# Autodesk Inventor assembly: Bridge
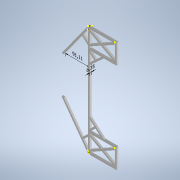
[picture p0: Inventor's stored thumbnail of the model, 180x180]
Saved by Autodesk Inventor 2020.1 (Build 241239000, 239)
## iProperties
Created: 2020-02-04
Part Number: Bridge
Document SubType Name: Assembly
Designer: super
Author: super
## Documents named in this file (8)
- C:\Users\super\Desktop\Giovanni\Science\3D Models\Autodesk-Inventor\Projects\FAS\Bridge.iam
- C:\Users\super\Desktop\Giovanni\Science\3D Models\Autodesk-Inventor\Projects\FAS\BottomBottom.ipt
- C:\Users\super\Desktop\Giovanni\Science\3D Models\Autodesk-Inventor\Projects\FAS\BottomDiagonalSupport.ipt
- C:\Users\super\Desktop\Giovanni\Science\3D Models\Autodesk-Inventor\Projects\FAS\BottomSquareSupport.ipt
- C:\Users\super\Desktop\Giovanni\Science\3D Models\Autodesk-Inventor\Projects\FAS\InnerDiagonalSupport.ipt
- C:\Users\super\Desktop\Giovanni\Science\3D Models\Autodesk-Inventor\Projects\FAS\Main.ipt
- C:\Users\super\Desktop\Giovanni\Science\3D Models\Autodesk-Inventor\Projects\FAS\UpperExteriorDiagonal.ipt
- C:\Users\super\Desktop\Giovanni\Science\3D Models\Autodesk-Inventor\Projects\FAS\UpperMiniSupport.ipt
## Components (19 placed, 7 different names)
1. BottomBottom:1 — Mate:1, Flush:1, Flush:2, Flush:3, Mate:2, Flush:4, Mate:3, Flush:5, Mate:4, Mate:5, Flush:6, Flush:15, Mate:12
2. BottomDiagonalSupport:1 — Mate:3, Flush:7, Mate:12, Rigid:3, Flush:20, Flush:21, Flush:22, Flush:23
3. BottomSquareSupport:1 — Mate:1, Flush:1, Flush:2, Flush:16, Flush:17, Rigid:3, Flush:20, Flush:23, Flush:24
4. BottomSquareSupport:2 — Flush:3, Mate:2, Flush:4, Rigid:1, Flush:19, Mate:16
5. BottomDiagonalSupport:2 — Flush:5, Mate:4, Rigid:1, Mate:5, Flush:6, Flush:7, Flush:21, Flush:22, Flush:24
6. BottomBottom:2 — Flush:15
7. BottomDiagonalSupport:3
8. BottomSquareSupport:3 — Mate:11, Mate:14
9. BottomSquareSupport:4 — Flush:18, Flush:19
10. BottomDiagonalSupport:4
11. Main:1 — Flush:16, Flush:17, Flush:18, Mate:11, Mate:13, Flush:25, Mate:15, Flush:26, Mate:17, Flush:27, Mate:18, Flush:28, Mate:19
12. InnerDiagonalSupport:1 — Mate:13, Mate:14, Flush:25
13. InnerDiagonalSupport:2 — Mate:15, Mate:16, Flush:26
14. UpperExteriorDiagonal:1 — Mate:17, Flush:27
15. UpperExteriorDiagonal:2 — Mate:18, Flush:28
16. UpperMiniSupport:1 — Mate:19
17. UpperMiniSupport:2
18. UpperMiniSupport:3
19. UpperMiniSupport:4
## Relationships (50: Flush 28, Mate 19, WeldJoint 3)
- Mate:1: BottomBottom:1 ↔ BottomSquareSupport:1
- Flush:1: BottomBottom:1 ↔ BottomSquareSupport:1
- Flush:2: BottomBottom:1 ↔ BottomSquareSupport:1
- Flush:3: BottomBottom:1 ↔ BottomSquareSupport:2
- Mate:2: BottomBottom:1 ↔ BottomSquareSupport:2
- Flush:4: BottomBottom:1 ↔ BottomSquareSupport:2
- Mate:3: BottomBottom:1 ↔ BottomDiagonalSupport:1
- Flush:5: BottomBottom:1 ↔ BottomDiagonalSupport:2
- Mate:4: BottomBottom:1 ↔ BottomDiagonalSupport:2
- Rigid:1 [WeldJoint]: BottomSquareSupport:2 ↔ BottomDiagonalSupport:2
- Mate:5: BottomBottom:1 ↔ BottomDiagonalSupport:2
- Flush:6: BottomBottom:1 ↔ BottomDiagonalSupport:2
- Flush:7: BottomDiagonalSupport:1 ↔ BottomDiagonalSupport:2
- [Mate]: BottomBottom:2 ↔ BottomSquareSupport:3
- [Flush]: BottomBottom:2 ↔ BottomSquareSupport:3
- [Flush]: BottomBottom:2 ↔ BottomSquareSupport:3
- [Flush]: BottomBottom:2 ↔ BottomSquareSupport:4
- [Mate]: BottomBottom:2 ↔ BottomSquareSupport:4
- [Flush]: BottomBottom:2 ↔ BottomSquareSupport:4
- [Mate]: BottomBottom:2 ↔ BottomDiagonalSupport:3
- [Flush]: BottomBottom:2 ↔ BottomDiagonalSupport:4
- [Mate]: BottomBottom:2 ↔ BottomDiagonalSupport:4
- [WeldJoint]: BottomSquareSupport:4 ↔ BottomDiagonalSupport:4
- [Mate]: BottomBottom:2 ↔ BottomDiagonalSupport:4
- [Flush]: BottomBottom:2 ↔ BottomDiagonalSupport:4
- [Flush]: BottomDiagonalSupport:3 ↔ BottomDiagonalSupport:4
- Flush:15: BottomBottom:1 ↔ BottomBottom:2
- Flush:16: BottomSquareSupport:1 ↔ Main:1
- Flush:17: BottomSquareSupport:1 ↔ Main:1
- Flush:18: BottomSquareSupport:4 ↔ Main:1
- Mate:11: BottomSquareSupport:3 ↔ Main:1
- Flush:19: BottomSquareSupport:2 ↔ BottomSquareSupport:4
- Mate:12: BottomBottom:1 ↔ BottomDiagonalSupport:1
- Rigid:3 [WeldJoint]: BottomDiagonalSupport:1 ↔ BottomSquareSupport:1
- Flush:20: BottomDiagonalSupport:1 ↔ BottomSquareSupport:1
- Flush:21: BottomDiagonalSupport:1 ↔ BottomDiagonalSupport:2
- Flush:22: BottomDiagonalSupport:1 ↔ BottomDiagonalSupport:2
- Flush:23: BottomDiagonalSupport:1 ↔ BottomSquareSupport:1
- Flush:24: BottomSquareSupport:1 ↔ BottomDiagonalSupport:2
- Mate:13: Main:1 ↔ InnerDiagonalSupport:1
- Mate:14: BottomSquareSupport:3 ↔ InnerDiagonalSupport:1
- Flush:25: Main:1 ↔ InnerDiagonalSupport:1
- Mate:15: Main:1 ↔ InnerDiagonalSupport:2
- Mate:16: BottomSquareSupport:2 ↔ InnerDiagonalSupport:2
- Flush:26: Main:1 ↔ InnerDiagonalSupport:2
- Mate:17: Main:1 ↔ UpperExteriorDiagonal:1
- Flush:27: Main:1 ↔ UpperExteriorDiagonal:1
- Mate:18: Main:1 ↔ UpperExteriorDiagonal:2
- Flush:28: Main:1 ↔ UpperExteriorDiagonal:2
- Mate:19: Main:1 ↔ UpperMiniSupport:1
## Named parameters: d13_d10 = 0 mm, d14_d11 = 0 mm, d15_d12 = 0 mm, d16_d1 = 0 mm, d17_d2 = 0 mm, d18_d3 = 0 mm, d19_d4 = 0 mm, d20_d5 = 0 mm, d21_d6 = 0 mm, d22_d7 = 0 mm, d23_d8 = 0 mm, d24_d9 = 0 mm, d25_d0 = 0 mm
